# Autodesk Inventor assembly: subflap2
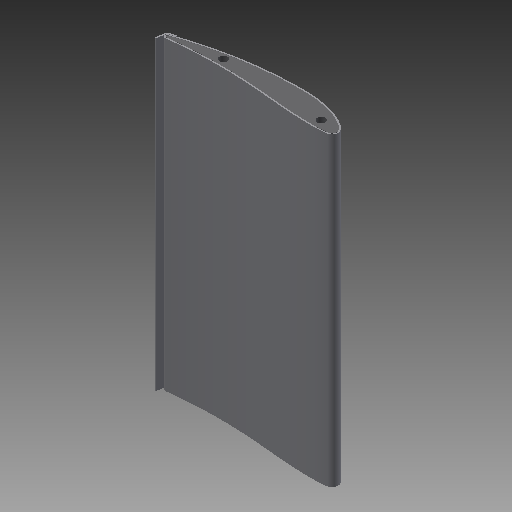
[picture p0: Inventor's stored thumbnail of the model, 512x512]
Saved by Autodesk Inventor 2018 (Build 220112000, 112)
## iProperties
Created: 2018-03-05
Part Number: subflap2
Material: 一般
Document SubType Name: Assembly
Designer: ku_sk
Author: ku_sk
## Documents named in this file (5)
- D:\Users\ku_sk\Documents\Inventor\Aero\KS-15\Fr.wing\parts\subflap\subflap.iam
- D:\Users\ku_sk\Documents\Inventor\Aero\KS-15\Fr.wing\parts\subflap\plate_sf.ipt
- D:\Users\ku_sk\Documents\Inventor\Aero\KS-15\Fr.wing\parts\subflap\uretan_sf.ipt
- D:\Users\ku_sk\Documents\Inventor\Aero\KS-15\Fr.wing\parts\subflap\GFRP_sf.ipt
- D:\Users\ku_sk\Documents\Inventor\Aero\KS-15\Fr.wing\parts\subflap\gurnee.ipt
## Components (13 placed, 4 different names)
1. plate_sf:1 — メイト:1, メイト:2, メイト:3, メイト:4, フラッシュ:2, メイト:5, メイト:14, メイト:15, メイト:16, メイト:17, フラッシュ:6
2. plate_sf:2 — フラッシュ:1, メイト:2, メイト:3, メイト:9, メイト:10, メイト:21, メイト:22
3. plate_sf:3 — フラッシュ:2, フラッシュ:3, メイト:5, メイト:6, メイト:13, メイト:14, メイト:18
4. plate_sf:4 — フラッシュ:3, フラッシュ:4, メイト:6, メイト:7, メイト:12, メイト:13, メイト:19, メイト:20, メイト:27, メイト:28
5. plate_sf:5 — フラッシュ:4, フラッシュ:5, メイト:7, メイト:8, メイト:11, メイト:12, メイト:25, メイト:26
6. plate_sf:6 — フラッシュ:5, メイト:8, メイト:9, メイト:10, メイト:11, メイト:23, メイト:24
7. uretan_sf:1 — メイト:21, メイト:22, メイト:23
8. uretan_sf:2 — メイト:24, メイト:25, メイト:26
9. uretan_sf:3 — メイト:27, メイト:28
10. uretan_sf:4 — メイト:18, メイト:19, メイト:20
11. uretan_sf:5 — メイト:15, メイト:16, メイト:17, メイト:29, メイト:30
12. GFRP_sf:1 — メイト:29, メイト:30, フラッシュ:6, メイト:31, フラッシュ:7, タッチ:1, タッチ:2
13. gurnee:1 — メイト:31, フラッシュ:7, タッチ:1, タッチ:2
## Relationships (40: Mate 31, Flush 7, Transitional 2)
- メイト:1 [Mate] (-110 mm): plate_sf:1
- フラッシュ:1 [Flush] (-115 mm): plate_sf:2
- メイト:2 [Mate]: plate_sf:1 ↔ plate_sf:2
- メイト:3 [Mate]: plate_sf:1 ↔ plate_sf:2
- メイト:4 [Mate]: plate_sf:1
- フラッシュ:2 [Flush] (-44.2 mm): plate_sf:1 ↔ plate_sf:3
- フラッシュ:3 [Flush] (-44.2 mm): plate_sf:3 ↔ plate_sf:4
- フラッシュ:4 [Flush] (-44.2 mm): plate_sf:4 ↔ plate_sf:5
- フラッシュ:5 [Flush] (-44.2 mm): plate_sf:5 ↔ plate_sf:6
- メイト:5 [Mate]: plate_sf:1 ↔ plate_sf:3
- メイト:6 [Mate]: plate_sf:3 ↔ plate_sf:4
- メイト:7 [Mate]: plate_sf:4 ↔ plate_sf:5
- メイト:8 [Mate]: plate_sf:5 ↔ plate_sf:6
- メイト:9 [Mate]: plate_sf:2 ↔ plate_sf:6
- メイト:10 [Mate]: plate_sf:2 ↔ plate_sf:6
- メイト:11 [Mate]: plate_sf:5 ↔ plate_sf:6
- メイト:12 [Mate]: plate_sf:4 ↔ plate_sf:5
- メイト:13 [Mate]: plate_sf:3 ↔ plate_sf:4
- メイト:14 [Mate]: plate_sf:1 ↔ plate_sf:3
- メイト:15 [Mate]: plate_sf:1 ↔ uretan_sf:5
- メイト:16 [Mate]: plate_sf:1 ↔ uretan_sf:5
- メイト:17 [Mate]: plate_sf:1 ↔ uretan_sf:5
- メイト:18 [Mate]: plate_sf:3 ↔ uretan_sf:4
- メイト:19 [Mate]: plate_sf:4 ↔ uretan_sf:4
- メイト:20 [Mate]: plate_sf:4 ↔ uretan_sf:4
- メイト:21 [Mate]: plate_sf:2 ↔ uretan_sf:1
- メイト:22 [Mate]: plate_sf:2 ↔ uretan_sf:1
- メイト:23 [Mate]: plate_sf:6 ↔ uretan_sf:1
- メイト:24 [Mate]: plate_sf:6 ↔ uretan_sf:2
- メイト:25 [Mate]: plate_sf:5 ↔ uretan_sf:2
- メイト:26 [Mate]: plate_sf:5 ↔ uretan_sf:2
- メイト:27 [Mate]: plate_sf:4 ↔ uretan_sf:3
- メイト:28 [Mate]: plate_sf:4 ↔ uretan_sf:3
- メイト:29 [Mate]: uretan_sf:5 ↔ GFRP_sf:1
- メイト:30 [Mate]: uretan_sf:5 ↔ GFRP_sf:1
- フラッシュ:6 [Flush]: plate_sf:1 ↔ GFRP_sf:1
- メイト:31 [Mate]: GFRP_sf:1 ↔ gurnee:1
- フラッシュ:7 [Flush]: GFRP_sf:1 ↔ gurnee:1
- タッチ:1 [Transitional]: GFRP_sf:1 ↔ gurnee:1
- タッチ:2 [Transitional]: GFRP_sf:1 ↔ gurnee:1
